# Autodesk Inventor assembly: mg996r_top_two_servo_v1
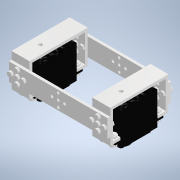
[picture p0: Inventor's stored thumbnail of the model, 180x180]
Saved by Autodesk Inventor 2021.4 (Build 254397000, 397)
## iProperties
Created: 2022-07-25
Part Number: mg996r_top_two_servo_v1
Document SubType Name: Assembly
Designer: isamu
Author: isamu
## Documents named in this file (5)
- D:\personal_projects\robot\inventor\2021_matlab_compat\mg996r_top_two_servo_v1.iam
- D:\personal_projects\robot\inventor\2021_matlab_compat\mg996r_servo_frame.iam
- D:\personal_projects\robot\exports\frames\servo frame part 4.ipt
- D:\personal_projects\robot\exports\screws\m3x8.ipt
- D:\personal_projects\robot\exports\screws\m3 nuts.ipt
## Components (44 placed, 4 different names)
1. mg996r_servo_frame:1 [sub-assembly] — Mate:1, Mate:2, Mate:3, Mate:10, Mate:11, Insert:21, Insert:22, Insert:23, Insert:24, Insert:25, Insert:31, Insert:32, Insert:33, Insert:34, Insert:35
2. mg996r_servo_frame:2 [sub-assembly] — Mate:4, Mate:5, Mate:6, Mate:7, Mate:8, Mate:9, Insert:26, Insert:27, Insert:28, Insert:29, Insert:30, Insert:36, Insert:37, Insert:38, Insert:39, Insert:40
3. servo frame part 4:1 — Mate:1, Mate:2, Mate:3, Mate:4, Mate:5, Mate:6, Insert:11, Insert:12, Insert:13, Insert:14, Insert:15, Insert:16, Insert:17, Insert:18, Insert:19, Insert:20
4. servo frame part 4:2 — Mate:7, Mate:8, Mate:9, Mate:10, Mate:11, Insert:1, Insert:2, Insert:3, Insert:4, Insert:5, Insert:6, Insert:7, Insert:8, Insert:9, Insert:10
5. m3x8:1 — Insert:4
6. m3x8:2 — Insert:3
7. m3x8:3 — Insert:5
8. m3x8:4 — Insert:14
9. m3x8:5 — Insert:17
10. m3x8:6 — Insert:15
11. m3x8:7 — Insert:11
12. m3x8:8 — Insert:12
13. m3x8:9 — Insert:13
14. m3x8:10 — Insert:16
15. m3x8:11 — Insert:7
16. m3x8:12 — Insert:10
17. m3x8:13 — Insert:19
18. m3x8:14 — Insert:20
19. m3x8:15 — Insert:6
20. m3x8:16 — Insert:1
21. m3x8:17 — Insert:2
22. m3x8:18 — Insert:8
23. m3x8:19 — Insert:9
24. m3x8:20 — Insert:18
25. m3 nuts:1 — Insert:31
26. m3 nuts:2 — Insert:29
27. m3 nuts:3 — Insert:23
28. m3 nuts:4 — Insert:22
29. m3 nuts:5 — Insert:21
30. m3 nuts:6 — Insert:32
31. m3 nuts:7 — Insert:33
32. m3 nuts:8 — Insert:36
33. m3 nuts:9 — Insert:39
34. m3 nuts:10 — Insert:35
35. m3 nuts:11 — Insert:34
36. m3 nuts:12 — Insert:30
37. m3 nuts:13 — Insert:24
38. m3 nuts:14 — Insert:28
39. m3 nuts:15 — Insert:25
40. m3 nuts:16 — Insert:38
41. m3 nuts:17 — Insert:40
42. m3 nuts:18 — Insert:37
43. m3 nuts:19 — Insert:27
44. m3 nuts:20 — Insert:26
## Relationships (51: Insert 40, Mate 11)
- Mate:1: mg996r_servo_frame:1 ↔ servo frame part 4:1
- Mate:2: mg996r_servo_frame:1 ↔ servo frame part 4:1
- Mate:3: mg996r_servo_frame:1 ↔ servo frame part 4:1
- Mate:4: mg996r_servo_frame:2 ↔ servo frame part 4:1
- Mate:5: mg996r_servo_frame:2 ↔ servo frame part 4:1
- Mate:6: mg996r_servo_frame:2 ↔ servo frame part 4:1
- Mate:7: mg996r_servo_frame:2 ↔ servo frame part 4:2
- Mate:8: mg996r_servo_frame:2 ↔ servo frame part 4:2
- Mate:9: mg996r_servo_frame:2 ↔ servo frame part 4:2
- Mate:10: mg996r_servo_frame:1 ↔ servo frame part 4:2
- Mate:11: mg996r_servo_frame:1 ↔ servo frame part 4:2
- Insert:1: servo frame part 4:2 ↔ m3x8:16
- Insert:2: servo frame part 4:2 ↔ m3x8:17
- Insert:3: servo frame part 4:2 ↔ m3x8:2
- Insert:4: servo frame part 4:2 ↔ m3x8:1
- Insert:5: servo frame part 4:2 ↔ m3x8:3
- Insert:6: servo frame part 4:2 ↔ m3x8:15
- Insert:7: servo frame part 4:2 ↔ m3x8:11
- Insert:8: servo frame part 4:2 ↔ m3x8:18
- Insert:9: servo frame part 4:2 ↔ m3x8:19
- Insert:10: servo frame part 4:2 ↔ m3x8:12
- Insert:11: servo frame part 4:1 ↔ m3x8:7
- Insert:12: servo frame part 4:1 ↔ m3x8:8
- Insert:13: servo frame part 4:1 ↔ m3x8:9
- Insert:14: servo frame part 4:1 ↔ m3x8:4
- Insert:15: servo frame part 4:1 ↔ m3x8:6
- Insert:16: servo frame part 4:1 ↔ m3x8:10
- Insert:17: servo frame part 4:1 ↔ m3x8:5
- Insert:18: servo frame part 4:1 ↔ m3x8:20
- Insert:19: servo frame part 4:1 ↔ m3x8:13
- Insert:20: servo frame part 4:1 ↔ m3x8:14
- Insert:21: mg996r_servo_frame:1 ↔ m3 nuts:5
- Insert:22: mg996r_servo_frame:1 ↔ m3 nuts:4
- Insert:23: mg996r_servo_frame:1 ↔ m3 nuts:3
- Insert:24: mg996r_servo_frame:1 ↔ m3 nuts:13
- Insert:25: mg996r_servo_frame:1 ↔ m3 nuts:15
- Insert:26: mg996r_servo_frame:2 ↔ m3 nuts:20
- Insert:27: mg996r_servo_frame:2 ↔ m3 nuts:19
- Insert:28: mg996r_servo_frame:2 ↔ m3 nuts:14
- Insert:29: mg996r_servo_frame:2 ↔ m3 nuts:2
- Insert:30: mg996r_servo_frame:2 ↔ m3 nuts:12
- Insert:31: mg996r_servo_frame:1 ↔ m3 nuts:1
- Insert:32: mg996r_servo_frame:1 ↔ m3 nuts:6
- Insert:33: mg996r_servo_frame:1 ↔ m3 nuts:7
- Insert:34: mg996r_servo_frame:1 ↔ m3 nuts:11
- Insert:35: mg996r_servo_frame:1 ↔ m3 nuts:10
- Insert:36: mg996r_servo_frame:2 ↔ m3 nuts:8
- Insert:37: mg996r_servo_frame:2 ↔ m3 nuts:18
- Insert:38: mg996r_servo_frame:2 ↔ m3 nuts:16
- Insert:39: mg996r_servo_frame:2 ↔ m3 nuts:9
- Insert:40: mg996r_servo_frame:2 ↔ m3 nuts:17
